# Autodesk Inventor assembly: Ensamblaje de Impresion 3D
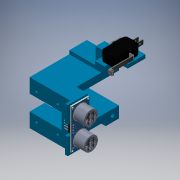
[picture p0: Inventor's stored thumbnail of the model, 180x180]
Saved by Autodesk Inventor 2018.3 (Build 223284000, 284)
## iProperties
Created: 2020-12-15
Part Number: Ensamblaje de Impresion 3D
Material: Genérico
Document SubType Name: Assembly
Designer: SERGIO ROMO
Author: SERGIO ROMO
## Documents named in this file (4)
- C:\Users\SERGIO ROMO\Documents\GitHub\RemBot\CAD\Balanceo de masa\Inventor\Ensamblaje de Impresion 3D.iam
- C:\Users\SERGIO ROMO\Documents\GitHub\RemBot\CAD\Balanceo de masa\Inventor\Impresion3D.ipt
- C:\Users\SERGIO ROMO\Documents\GitHub\RemBot\CAD\Balanceo de masa\Inventor\KW8-2.ipt
- C:\Users\SERGIO ROMO\Documents\GitHub\RemBot\CAD\Balanceo de masa\Inventor\HC-SR04 Ultrasonico.iam
## Components (3 placed, 3 different names)
1. Impresion3D:1 — De rotación:1
2. KW8-2:1
3. HC-SR04 Ultrasonico:1 [sub-assembly] — De rotación:1
## Relationships (1: RevoluteJoint 1)
- De rotación:1 [RevoluteJoint]: Impresion3D:1 ↔ HC-SR04 Ultrasonico:1
